# Autodesk Inventor assembly: Gripper_Design_Non_Compliant_v1
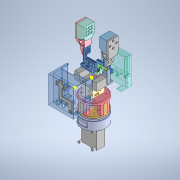
[picture p0: Inventor's stored thumbnail of the model, 180x180]
Saved by Autodesk Inventor 2022 (Build 260153000, 153)
## iProperties
Created: 2021-07-25
Part Number: Gripper_Design_Non_Compliant_v1
Document SubType Name: Assembly
Designer: exllu
Author: exllu
## Documents named in this file (36)
- C:\Users\kylem\OneDrive\Documents\1 - Documents\Gripper Design\Gripper_Design_Non_Compliant_v1.iam
- C:\Users\kylem\OneDrive\Documents\1 - Documents\Gripper Design\Motor_XM,H-430_idler.ipt
- C:\Users\kylem\OneDrive\Documents\1 - Documents\Gripper Design\Carriage_8381K550.iam
- C:\Users\kylem\OneDrive\Documents\1 - Documents\Gripper Design\Rail_8381K550.iam
- C:\Users\kylem\OneDrive\Documents\1 - Documents\Gripper Design\Pinion_2664N316.ipt
- C:\Users\kylem\OneDrive\Documents\1 - Documents\Gripper Design\Drive_shaft.ipt
- C:\Users\kylem\OneDrive\Documents\1 - Documents\Gripper Design\Motor_horn_mount.ipt
- C:\Users\kylem\OneDrive\Documents\1 - Documents\Gripper Design\Rack.iam
- C:\Users\kylem\OneDrive\Documents\1 - Documents\Gripper Design\UR5 Robot\End-effector-plate.ipt
- C:\Users\kylem\OneDrive\Documents\1 - Documents\Gripper Design\Rail_lock_washer.ipt
- C:\Users\exllu\Downloads\Rail_nut.ipt
- C:\Users\exllu\Downloads\90910A901_Button Head Torx Screws.ipt
- C:\Users\kylem\OneDrive\Documents\1 - Documents\Gripper Design\Rail_screws.ipt
- C:\Users\kylem\OneDrive\Documents\1 - Documents\Gripper Design\Rail_mount.ipt
- C:\Users\kylem\OneDrive\Documents\1 - Documents\Gripper Design\Front_plate.ipt
- C:\Users\exllu\Downloads\UR5_Screws.ipt
- C:\Users\kylem\OneDrive\Documents\1 - Documents\Gripper Design\UR5_Mounting_Plate.ipt
- C:\Users\kylem\OneDrive\Documents\1 - Documents\Gripper Design\Motor_UR5_mount.ipt
- C:\Users\kylem\OneDrive\Documents\1 - Documents\Gripper Design\Cover_bottom.ipt
- C:\Users\kylem\OneDrive\Documents\1 - Documents\Gripper Design\Cover_top.ipt
- C:\Users\kylem\OneDrive\Documents\1 - Documents\Gripper Design\Non_compliant_plate.ipt
- C:\Users\kylem\OneDrive\Documents\1 - Documents\Gripper Design\Cover_bottom_raceway_cover.ipt
- C:\Users\exllu\Downloads\98689A110_ METRIC GENERAL PURPOSE WASHERS.ipt
- C:\Users\exllu\Downloads\91292A004_TYPE 18-8 SS SOCKET HEAD CAP SCREW.ipt
- C:\Users\exllu\Downloads\98689A112_ METRIC GENERAL PURPOSE WASHERS.ipt
- C:\Users\exllu\Downloads\92855A309_18-8 Stainless Steel Low-Profile Socket Head Screws.ipt
- C:\Users\exllu\Downloads\97163A149_TAPERED HEAT-SET INSERTS FOR PLASTIC .ipt
- C:\Users\exllu\Downloads\91223A411_316 SS ULTRA-LOW-PROFILE SOCKET HEAD SCREW.ipt
- C:\Users\exllu\Downloads\91290A099_Black-Oxide Alloy Steel Socket Head Screw.ipt
- C:\Users\exllu\Downloads\91292A834_TYPE 18-8 SS SOCKET HEAD CAP SCREW.ipt
- C:\Users\exllu\Downloads\91292A016_TYPE 18-8 SS SOCKET HEAD CAP SCREW.ipt
- C:\Users\exllu\Downloads\91292A022_18-8 Stainless Steel Socket Head Screw.ipt
- C:\Users\exllu\Downloads\97400A135_18-8 STAINLESS STEEL SERRATED FLANGE LOCKNUT.ipt
- C:\Users\kylem\OneDrive\Documents\1 - Documents\Gripper Design\U2D2PHB_Board.ipt
- C:\Users\kylem\OneDrive\Documents\1 - Documents\Gripper Design\Finger Assembly Left.iam
- C:\Users\kylem\OneDrive\Documents\1 - Documents\Gripper Design\Finger Assembly Right.iam
## Components (86 placed, 35 different names)
1. Motor_XM,H-430_idler:1 — Flush:1, Flush:2, Flush:3, Flush:7, Mate:15, Mate:16, Mate:29, Flush:22, Mate:65, Flush:33, Flush:34, Mate:132, Mate:218, Mate:238
2. Rail_8381K550:3 [sub-assembly] — Mate:3, Mate:4, Mate:5, Mate:6, Flush:7, Mate:29, Mate:30, Flush:18, Flush:19, Mate:36, Mate:40, Mate:41, Mate:44, Mate:45, Mate:47, Mate:53, Mate:55, Mate:56, Mate:57, Mate:59, Mate:61, Mate:62, Flush:25
3. Rail_8381K550:4 [sub-assembly] — Mate:1, Mate:2, Mate:7, Mate:8, Mate:30, Flush:18, Flush:19, Mate:32, Mate:33, Mate:34, Mate:35, Mate:37, Mate:38, Mate:39, Mate:46, Mate:63
4. Carriage_8381K550:5 [sub-assembly] — Mate:4, Mate:5, Flush:12, Mate:137, Mate:138, Mate:139, Mate:142
5. Carriage_8381K550:6 [sub-assembly] — Mate:1, Mate:7, Mate:13, Mate:140, Mate:143
6. Carriage_8381K550:7 [sub-assembly] — Mate:3, Mate:6, Mate:142
7. Carriage_8381K550:8 [sub-assembly] — Mate:2, Mate:8, Mate:13, Flush:23, Mate:141
8. Pinion_2664N316:1 — Mate:20, Mate:21, Flush:20, Tangent:1, Tangent:2, Rotation/Translation:1, Rotation/Translation:2, Mate:240
9. Drive_shaft:1 — Mate:17, Mate:20, Mate:21, Mate:66, Mate:220, Mate:221
10. Motor_horn_mount:1 — Mate:15, Mate:16, Mate:17, Mate:64, Mate:66
11. Rack:1 [sub-assembly] — Flush:20, Tangent:1, Flush:23, Rotation/Translation:2, Mate:190, Mate:191, Mate:192
12. Rack:2 [sub-assembly] — Flush:12, Tangent:2, Rotation/Translation:1, Mate:182, Mate:185, Mate:186
13. End-effector-plate:1 — Flush:33, Flush:34, Mate:111, Mate:126, Mate:133
14. Rail_lock_washer:1 — Mate:40, Mate:41, Mate:52
15. Rail_nut:1 — Mate:32, Mate:39
16. Rail_nut:2 — Mate:33, Mate:38
17. Rail_lock_washer:3 — Mate:44, Mate:47, Mate:54
18. Rail_nut:3 — Mate:34, Mate:37
19. Rail_lock_washer:4 — Mate:45, Mate:46, Mate:60
20. Rail_nut:4 — Mate:35, Mate:36
21. 90910A901_Button Head Torx Screws:1 — Mate:52, Mate:53
22. Rail_screws:1 — Mate:60, Mate:61
23. Rail_screws:2 — Mate:54, Mate:55
24. Rail_screws:3 — Mate:58, Mate:59
25. Rail_lock_washer:5 — Mate:56, Mate:57, Mate:58
26. Rail_mount:1 — Mate:62, Mate:63, Flush:25, Mate:68, Mate:135, Mate:209
27. Front_plate:1 — Flush:22, Mate:64, Mate:65, Mate:68, Mate:210, Mate:222, Mate:223, Mate:240
28. UR5_Screws:1 — Mate:114, Mate:115
29. UR5_Screws:3 — Mate:118, Mate:122
30. UR5_Screws:4 — Mate:112, Mate:124
31. UR5_Mounting_Plate:1 — Mate:111, Mate:112, Mate:114, Mate:115, Mate:118, Mate:122, Mate:124, Mate:126, Mate:127, Mate:128, Mate:129, Mate:131, Mate:133
32. Motor_UR5_mount:1 — Mate:129, Mate:131, Mate:132, Mate:134, Mate:136, Mate:224, Mate:225, Mate:228, Mate:229, Mate:232, Mate:234, Mate:236, Mate:237
33. UR5_Screws:5 — Mate:127, Mate:128
34. Cover_bottom:1 — Mate:134, Mate:135, Flush:35, Mate:145, Flush:36, Mate:146, Flush:41, Mate:214, Mate:239
35. Cover_top:1 — Mate:136, Flush:35, Mate:216, Mate:217, Mate:219
36. Non_compliant_plate:1 — Mate:140, Mate:141, Mate:143, Mate:155, Mate:156, Mate:157, Mate:158, Mate:159, Mate:160, Mate:161, Mate:162, Mate:173, Mate:174, Mate:175, Mate:176, Mate:187, Mate:188, Mate:189, Mate:207, Mate:208, Flush:39, Flush:40, Mate:242, Flush:42, Mate:244
37. Non_compliant_plate:2 — Mate:137, Mate:138, Mate:139, Mate:147, Mate:148, Mate:149, Mate:150, Mate:151, Mate:152, Mate:153, Mate:154, Mate:177, Mate:178, Mate:179, Mate:180, Mate:181, Mate:183, Mate:184, Mate:205, Mate:206, Flush:37, Flush:38, Mate:241, Flush:43, Mate:243
38. Cover_bottom_raceway_cover:1 — Mate:145, Flush:36, Mate:146, Mate:211, Mate:212
39. 98689A110_ METRIC GENERAL PURPOSE WASHERS:1 — Mate:149, Mate:152, Mate:166
40. 98689A110_ METRIC GENERAL PURPOSE WASHERS:2 — Mate:158, Mate:159, Mate:172
41. 98689A110_ METRIC GENERAL PURPOSE WASHERS:3 — Mate:156, Mate:161, Mate:170
42. 98689A110_ METRIC GENERAL PURPOSE WASHERS:4 — Mate:157, Mate:160, Mate:171
43. 98689A110_ METRIC GENERAL PURPOSE WASHERS:5 — Mate:155, Mate:162, Mate:169
44. 98689A110_ METRIC GENERAL PURPOSE WASHERS:6 — Mate:150, Mate:151, Mate:165
45. 98689A110_ METRIC GENERAL PURPOSE WASHERS:7 — Mate:147, Mate:154, Mate:168
46. 98689A110_ METRIC GENERAL PURPOSE WASHERS:8 — Mate:148, Mate:153, Mate:167
47. 91292A004_TYPE 18-8 SS SOCKET HEAD CAP SCREW:1 — Mate:168, Mate:180
48. 91292A004_TYPE 18-8 SS SOCKET HEAD CAP SCREW:2 — Mate:166, Mate:178
49. 91292A004_TYPE 18-8 SS SOCKET HEAD CAP SCREW:3 — Mate:165, Mate:177
50. 91292A004_TYPE 18-8 SS SOCKET HEAD CAP SCREW:4 — Mate:167, Mate:179
51. 91292A004_TYPE 18-8 SS SOCKET HEAD CAP SCREW:5 — Mate:171, Mate:174
52. 91292A004_TYPE 18-8 SS SOCKET HEAD CAP SCREW:6 — Mate:169, Mate:176
53. 91292A004_TYPE 18-8 SS SOCKET HEAD CAP SCREW:7 — Mate:172, Mate:173
54. 91292A004_TYPE 18-8 SS SOCKET HEAD CAP SCREW:8 — Mate:170, Mate:175
55. 98689A112_ METRIC GENERAL PURPOSE WASHERS:1 — Mate:181, Mate:182, Mate:193, Mate:204
56. 98689A112_ METRIC GENERAL PURPOSE WASHERS:2 — Mate:189, Mate:191, Mate:197, Mate:200
57. 98689A112_ METRIC GENERAL PURPOSE WASHERS:3 — Mate:188, Mate:190, Mate:196, Mate:201
58. 98689A112_ METRIC GENERAL PURPOSE WASHERS:4 — Mate:187, Mate:192, Mate:198, Mate:199
59. 98689A112_ METRIC GENERAL PURPOSE WASHERS:6 — Mate:184, Mate:186, Mate:195, Mate:202
60. 98689A112_ METRIC GENERAL PURPOSE WASHERS:7 — Mate:183, Mate:185, Mate:194, Mate:203
61. 92855A309_18-8 Stainless Steel Low-Profile Socket Head Screws:1 — Mate:195, Mate:202
62. 92855A309_18-8 Stainless Steel Low-Profile Socket Head Screws:2 — Mate:198, Mate:199
63. 92855A309_18-8 Stainless Steel Low-Profile Socket Head Screws:3 — Mate:194, Mate:203
64. 92855A309_18-8 Stainless Steel Low-Profile Socket Head Screws:4 — Mate:197, Mate:200
65. 92855A309_18-8 Stainless Steel Low-Profile Socket Head Screws:5 — Mate:193, Mate:204
66. 92855A309_18-8 Stainless Steel Low-Profile Socket Head Screws:6 — Mate:196, Mate:201
67. 97163A149_TAPERED HEAT-SET INSERTS FOR PLASTIC :1 — Mate:205, Flush:38
68. 97163A149_TAPERED HEAT-SET INSERTS FOR PLASTIC :2 — Mate:206, Flush:37
69. 97163A149_TAPERED HEAT-SET INSERTS FOR PLASTIC :3 — Mate:207, Flush:40
70. 97163A149_TAPERED HEAT-SET INSERTS FOR PLASTIC :4 — Mate:208, Flush:39
71. 92855A309_18-8 Stainless Steel Low-Profile Socket Head Screws:7 — Mate:209, Mate:210
72. 91223A411_316 SS ULTRA-LOW-PROFILE SOCKET HEAD SCREW:1 — Mate:211, Mate:212
73. 97163A149_TAPERED HEAT-SET INSERTS FOR PLASTIC :5 — Flush:41, Mate:214
74. 92855A309_18-8 Stainless Steel Low-Profile Socket Head Screws:8 — Mate:216, Mate:217
75. 91290A099_Black-Oxide Alloy Steel Socket Head Screw:1 — Mate:218, Mate:219
76. 91292A834_TYPE 18-8 SS SOCKET HEAD CAP SCREW:1 — Mate:220, Mate:221
77. 91292A016_TYPE 18-8 SS SOCKET HEAD CAP SCREW:1 — Mate:222, Mate:223
78. 91292A022_18-8 Stainless Steel Socket Head Screw:1 — Mate:224, Mate:225, Mate:233
79. 91292A022_18-8 Stainless Steel Socket Head Screw:2 — Mate:228, Mate:229, Mate:235
80. 97400A135_18-8 STAINLESS STEEL SERRATED FLANGE LOCKNUT:1 — Mate:232, Mate:233
81. 97400A135_18-8 STAINLESS STEEL SERRATED FLANGE LOCKNUT:2 — Mate:234, Mate:235
82. 91292A016_TYPE 18-8 SS SOCKET HEAD CAP SCREW:2 — Mate:236, Mate:237
83. 91290A099_Black-Oxide Alloy Steel Socket Head Screw:2 — Mate:238, Mate:239
84. U2D2PHB_Board:1
85. Finger Assembly Left:1 [sub-assembly] — Mate:241, Flush:43, Mate:243
86. Finger Assembly Right:1 [sub-assembly] — Mate:242, Flush:42, Mate:244
## Relationships (188: Mate 162, Flush 22, Tangent 2, RelateRotateTranslate 2)
- Mate:1 (0.1 mm): Rail_8381K550:4 ↔ Carriage_8381K550:6
- Mate:2 (0.1 mm): Rail_8381K550:4 ↔ Carriage_8381K550:8
- Mate:3 (0.1 mm): Rail_8381K550:3 ↔ Carriage_8381K550:7
- Mate:4 (0.1 mm): Rail_8381K550:3 ↔ Carriage_8381K550:5
- Mate:5 (0.2 mm): Rail_8381K550:3 ↔ Carriage_8381K550:5
- Mate:6 (0.2 mm): Rail_8381K550:3 ↔ Carriage_8381K550:7
- Mate:7 (0.2 mm): Rail_8381K550:4 ↔ Carriage_8381K550:6
- Mate:8 (0.2 mm): Rail_8381K550:4 ↔ Carriage_8381K550:8
- Flush:1: Motor_XM,H-430_idler:1
- Flush:2: Motor_XM,H-430_idler:1
- Flush:3: Motor_XM,H-430_idler:1
- Mate:13: Carriage_8381K550:6 ↔ Carriage_8381K550:8
- Flush:7 (-20.75 mm): Motor_XM,H-430_idler:1 ↔ Rail_8381K550:3
- Mate:15: Motor_XM,H-430_idler:1 ↔ Motor_horn_mount:1
- Mate:16: Motor_XM,H-430_idler:1 ↔ Motor_horn_mount:1
- Mate:17: Drive_shaft:1 ↔ Motor_horn_mount:1
- Mate:20: Pinion_2664N316:1 ↔ Drive_shaft:1
- Mate:21: Pinion_2664N316:1 ↔ Drive_shaft:1
- Flush:12: Carriage_8381K550:5 ↔ Rack:2
- Mate:29 (-10.75 mm): Motor_XM,H-430_idler:1 ↔ Rail_8381K550:3
- Mate:30 (1 mm): Rail_8381K550:3 ↔ Rail_8381K550:4
- Flush:18: Rail_8381K550:3 ↔ Rail_8381K550:4
- Flush:19: Rail_8381K550:3 ↔ Rail_8381K550:4
- Flush:20: Pinion_2664N316:1 ↔ Rack:1
- Mate:32: Rail_8381K550:4 ↔ Rail_nut:1
- Mate:33: Rail_8381K550:4 ↔ Rail_nut:2
- Mate:34: Rail_8381K550:4 ↔ Rail_nut:3
- Mate:35: Rail_8381K550:4 ↔ Rail_nut:4
- Mate:36: Rail_8381K550:3 ↔ Rail_nut:4
- Mate:37: Rail_8381K550:4 ↔ Rail_nut:3
- Mate:38: Rail_8381K550:4 ↔ Rail_nut:2
- Mate:39: Rail_8381K550:4 ↔ Rail_nut:1
- Mate:40: Rail_8381K550:3 ↔ Rail_lock_washer:1
- Mate:41: Rail_8381K550:3 ↔ Rail_lock_washer:1
- Mate:44: Rail_8381K550:3 ↔ Rail_lock_washer:3
- Mate:45: Rail_8381K550:3 ↔ Rail_lock_washer:4
- Mate:46: Rail_8381K550:4 ↔ Rail_lock_washer:4
- Mate:47: Rail_8381K550:3 ↔ Rail_lock_washer:3
- Mate:52: Rail_lock_washer:1 ↔ 90910A901_Button Head Torx Screws:1
- Mate:53: Rail_8381K550:3 ↔ 90910A901_Button Head Torx Screws:1
- Mate:54: Rail_lock_washer:3 ↔ Rail_screws:2
- Mate:55: Rail_8381K550:3 ↔ Rail_screws:2
- Mate:56: Rail_8381K550:3 ↔ Rail_lock_washer:5
- Mate:57: Rail_8381K550:3 ↔ Rail_lock_washer:5
- Mate:58: Rail_screws:3 ↔ Rail_lock_washer:5
- Mate:59: Rail_8381K550:3 ↔ Rail_screws:3
- Mate:60: Rail_lock_washer:4 ↔ Rail_screws:1
- Mate:61: Rail_8381K550:3 ↔ Rail_screws:1
- Mate:62: Rail_8381K550:3 ↔ Rail_mount:1
- Mate:63: Rail_8381K550:4 ↔ Rail_mount:1
- Flush:22: Motor_XM,H-430_idler:1 ↔ Front_plate:1
- Mate:64: Motor_horn_mount:1 ↔ Front_plate:1
- Mate:65: Motor_XM,H-430_idler:1 ↔ Front_plate:1
- Tangent:1 (-1 mm): Pinion_2664N316:1 ↔ Rack:1
- Tangent:2 (-1 mm): Pinion_2664N316:1 ↔ Rack:2
- Rotation/Translation:1 [RelateRotateTranslate] (39.841 mm): Pinion_2664N316:1 ↔ Rack:2
- Mate:66: Drive_shaft:1 ↔ Motor_horn_mount:1
- Flush:23: Carriage_8381K550:8 ↔ Rack:1
- Flush:25: Rail_8381K550:3 ↔ Rail_mount:1
- Mate:68: Rail_mount:1 ↔ Front_plate:1
- Rotation/Translation:2 [RelateRotateTranslate] (40.841 mm): Pinion_2664N316:1 ↔ Rack:1
- Flush:33 (4.572 mm): Motor_XM,H-430_idler:1 ↔ End-effector-plate:1
- Flush:34 (15.25 mm): Motor_XM,H-430_idler:1 ↔ End-effector-plate:1
- Mate:111: End-effector-plate:1 ↔ UR5_Mounting_Plate:1
- Mate:112: UR5_Screws:4 ↔ UR5_Mounting_Plate:1
- Mate:114: UR5_Screws:1 ↔ UR5_Mounting_Plate:1
- Mate:115: UR5_Screws:1 ↔ UR5_Mounting_Plate:1
- Mate:118: UR5_Screws:3 ↔ UR5_Mounting_Plate:1
- Mate:122: UR5_Screws:3 ↔ UR5_Mounting_Plate:1
- Mate:124: UR5_Screws:4 ↔ UR5_Mounting_Plate:1
- Mate:126: End-effector-plate:1 ↔ UR5_Mounting_Plate:1
- Mate:127: UR5_Mounting_Plate:1 ↔ UR5_Screws:5
- Mate:128: UR5_Mounting_Plate:1 ↔ UR5_Screws:5
- Mate:129: UR5_Mounting_Plate:1 ↔ Motor_UR5_mount:1
- Mate:131: UR5_Mounting_Plate:1 ↔ Motor_UR5_mount:1
- Mate:132: Motor_XM,H-430_idler:1 ↔ Motor_UR5_mount:1
- Mate:133: End-effector-plate:1 ↔ UR5_Mounting_Plate:1
- Mate:134: Motor_UR5_mount:1 ↔ Cover_bottom:1
- Mate:135 (0.5 mm): Rail_mount:1 ↔ Cover_bottom:1
- Mate:136: Motor_UR5_mount:1 ↔ Cover_top:1
- Flush:35: Cover_bottom:1 ↔ Cover_top:1
- Mate:137: Carriage_8381K550:5 ↔ Non_compliant_plate:2
- Mate:138: Carriage_8381K550:5 ↔ Non_compliant_plate:2
- Mate:139: Carriage_8381K550:5 ↔ Non_compliant_plate:2
- Mate:140: Carriage_8381K550:6 ↔ Non_compliant_plate:1
- Mate:141: Carriage_8381K550:8 ↔ Non_compliant_plate:1
- Mate:142: Carriage_8381K550:5 ↔ Carriage_8381K550:7
- Mate:143: Carriage_8381K550:6 ↔ Non_compliant_plate:1
- Mate:145: Cover_bottom:1 ↔ Cover_bottom_raceway_cover:1
- Flush:36: Cover_bottom:1 ↔ Cover_bottom_raceway_cover:1
- Mate:146: Cover_bottom:1 ↔ Cover_bottom_raceway_cover:1
- Mate:147: Non_compliant_plate:2 ↔ 98689A110_ METRIC GENERAL PURPOSE WASHERS:7
- Mate:148: Non_compliant_plate:2 ↔ 98689A110_ METRIC GENERAL PURPOSE WASHERS:8
- Mate:149: Non_compliant_plate:2 ↔ 98689A110_ METRIC GENERAL PURPOSE WASHERS:1
- Mate:150: Non_compliant_plate:2 ↔ 98689A110_ METRIC GENERAL PURPOSE WASHERS:6
- Mate:151: Non_compliant_plate:2 ↔ 98689A110_ METRIC GENERAL PURPOSE WASHERS:6
- Mate:152: Non_compliant_plate:2 ↔ 98689A110_ METRIC GENERAL PURPOSE WASHERS:1
- Mate:153: Non_compliant_plate:2 ↔ 98689A110_ METRIC GENERAL PURPOSE WASHERS:8
- Mate:154: Non_compliant_plate:2 ↔ 98689A110_ METRIC GENERAL PURPOSE WASHERS:7
- Mate:155: Non_compliant_plate:1 ↔ 98689A110_ METRIC GENERAL PURPOSE WASHERS:5
- Mate:156: Non_compliant_plate:1 ↔ 98689A110_ METRIC GENERAL PURPOSE WASHERS:3
- Mate:157: Non_compliant_plate:1 ↔ 98689A110_ METRIC GENERAL PURPOSE WASHERS:4
- Mate:158: Non_compliant_plate:1 ↔ 98689A110_ METRIC GENERAL PURPOSE WASHERS:2
- Mate:159: Non_compliant_plate:1 ↔ 98689A110_ METRIC GENERAL PURPOSE WASHERS:2
- Mate:160: Non_compliant_plate:1 ↔ 98689A110_ METRIC GENERAL PURPOSE WASHERS:4
- Mate:161: Non_compliant_plate:1 ↔ 98689A110_ METRIC GENERAL PURPOSE WASHERS:3
- Mate:162: Non_compliant_plate:1 ↔ 98689A110_ METRIC GENERAL PURPOSE WASHERS:5
- Mate:165: 98689A110_ METRIC GENERAL PURPOSE WASHERS:6 ↔ 91292A004_TYPE 18-8 SS SOCKET HEAD CAP SCREW:3
- Mate:166: 98689A110_ METRIC GENERAL PURPOSE WASHERS:1 ↔ 91292A004_TYPE 18-8 SS SOCKET HEAD CAP SCREW:2
- Mate:167: 98689A110_ METRIC GENERAL PURPOSE WASHERS:8 ↔ 91292A004_TYPE 18-8 SS SOCKET HEAD CAP SCREW:4
- Mate:168: 98689A110_ METRIC GENERAL PURPOSE WASHERS:7 ↔ 91292A004_TYPE 18-8 SS SOCKET HEAD CAP SCREW:1
- Mate:169: 98689A110_ METRIC GENERAL PURPOSE WASHERS:5 ↔ 91292A004_TYPE 18-8 SS SOCKET HEAD CAP SCREW:6
- Mate:170: 98689A110_ METRIC GENERAL PURPOSE WASHERS:3 ↔ 91292A004_TYPE 18-8 SS SOCKET HEAD CAP SCREW:8
- Mate:171: 98689A110_ METRIC GENERAL PURPOSE WASHERS:4 ↔ 91292A004_TYPE 18-8 SS SOCKET HEAD CAP SCREW:5
- Mate:172: 98689A110_ METRIC GENERAL PURPOSE WASHERS:2 ↔ 91292A004_TYPE 18-8 SS SOCKET HEAD CAP SCREW:7
- Mate:173: Non_compliant_plate:1 ↔ 91292A004_TYPE 18-8 SS SOCKET HEAD CAP SCREW:7
- Mate:174: Non_compliant_plate:1 ↔ 91292A004_TYPE 18-8 SS SOCKET HEAD CAP SCREW:5
- Mate:175: Non_compliant_plate:1 ↔ 91292A004_TYPE 18-8 SS SOCKET HEAD CAP SCREW:8
- Mate:176: Non_compliant_plate:1 ↔ 91292A004_TYPE 18-8 SS SOCKET HEAD CAP SCREW:6
- Mate:177: Non_compliant_plate:2 ↔ 91292A004_TYPE 18-8 SS SOCKET HEAD CAP SCREW:3
- Mate:178: Non_compliant_plate:2 ↔ 91292A004_TYPE 18-8 SS SOCKET HEAD CAP SCREW:2
- Mate:179: Non_compliant_plate:2 ↔ 91292A004_TYPE 18-8 SS SOCKET HEAD CAP SCREW:4
- Mate:180: Non_compliant_plate:2 ↔ 91292A004_TYPE 18-8 SS SOCKET HEAD CAP SCREW:1
- Mate:181: Non_compliant_plate:2 ↔ 98689A112_ METRIC GENERAL PURPOSE WASHERS:1
- Mate:182: Rack:2 ↔ 98689A112_ METRIC GENERAL PURPOSE WASHERS:1
- Mate:183: Non_compliant_plate:2 ↔ 98689A112_ METRIC GENERAL PURPOSE WASHERS:7
- Mate:184: Non_compliant_plate:2 ↔ 98689A112_ METRIC GENERAL PURPOSE WASHERS:6
- Mate:185: Rack:2 ↔ 98689A112_ METRIC GENERAL PURPOSE WASHERS:7
- Mate:186: Rack:2 ↔ 98689A112_ METRIC GENERAL PURPOSE WASHERS:6
- Mate:187: Non_compliant_plate:1 ↔ 98689A112_ METRIC GENERAL PURPOSE WASHERS:4
- Mate:188: Non_compliant_plate:1 ↔ 98689A112_ METRIC GENERAL PURPOSE WASHERS:3
- Mate:189: Non_compliant_plate:1 ↔ 98689A112_ METRIC GENERAL PURPOSE WASHERS:2
- Mate:190: Rack:1 ↔ 98689A112_ METRIC GENERAL PURPOSE WASHERS:3
- Mate:191: Rack:1 ↔ 98689A112_ METRIC GENERAL PURPOSE WASHERS:2
- Mate:192: Rack:1 ↔ 98689A112_ METRIC GENERAL PURPOSE WASHERS:4
- Mate:193: 98689A112_ METRIC GENERAL PURPOSE WASHERS:1 ↔ 92855A309_18-8 Stainless Steel Low-Profile Socket Head Screws:5
- Mate:194: 98689A112_ METRIC GENERAL PURPOSE WASHERS:7 ↔ 92855A309_18-8 Stainless Steel Low-Profile Socket Head Screws:3
- Mate:195: 98689A112_ METRIC GENERAL PURPOSE WASHERS:6 ↔ 92855A309_18-8 Stainless Steel Low-Profile Socket Head Screws:1
- Mate:196: 98689A112_ METRIC GENERAL PURPOSE WASHERS:3 ↔ 92855A309_18-8 Stainless Steel Low-Profile Socket Head Screws:6
- Mate:197: 98689A112_ METRIC GENERAL PURPOSE WASHERS:2 ↔ 92855A309_18-8 Stainless Steel Low-Profile Socket Head Screws:4
- Mate:198: 98689A112_ METRIC GENERAL PURPOSE WASHERS:4 ↔ 92855A309_18-8 Stainless Steel Low-Profile Socket Head Screws:2
- Mate:199: 98689A112_ METRIC GENERAL PURPOSE WASHERS:4 ↔ 92855A309_18-8 Stainless Steel Low-Profile Socket Head Screws:2
- Mate:200: 98689A112_ METRIC GENERAL PURPOSE WASHERS:2 ↔ 92855A309_18-8 Stainless Steel Low-Profile Socket Head Screws:4
- Mate:201: 98689A112_ METRIC GENERAL PURPOSE WASHERS:3 ↔ 92855A309_18-8 Stainless Steel Low-Profile Socket Head Screws:6
- Mate:202: 98689A112_ METRIC GENERAL PURPOSE WASHERS:6 ↔ 92855A309_18-8 Stainless Steel Low-Profile Socket Head Screws:1
- Mate:203: 98689A112_ METRIC GENERAL PURPOSE WASHERS:7 ↔ 92855A309_18-8 Stainless Steel Low-Profile Socket Head Screws:3
- Mate:204: 98689A112_ METRIC GENERAL PURPOSE WASHERS:1 ↔ 92855A309_18-8 Stainless Steel Low-Profile Socket Head Screws:5
- Mate:205: Non_compliant_plate:2 ↔ 97163A149_TAPERED HEAT-SET INSERTS FOR PLASTIC :1
- Mate:206: Non_compliant_plate:2 ↔ 97163A149_TAPERED HEAT-SET INSERTS FOR PLASTIC :2
- Flush:37: Non_compliant_plate:2 ↔ 97163A149_TAPERED HEAT-SET INSERTS FOR PLASTIC :2
- Flush:38: Non_compliant_plate:2 ↔ 97163A149_TAPERED HEAT-SET INSERTS FOR PLASTIC :1
- Mate:207: Non_compliant_plate:1 ↔ 97163A149_TAPERED HEAT-SET INSERTS FOR PLASTIC :3
- Mate:208: Non_compliant_plate:1 ↔ 97163A149_TAPERED HEAT-SET INSERTS FOR PLASTIC :4
- Flush:39: Non_compliant_plate:1 ↔ 97163A149_TAPERED HEAT-SET INSERTS FOR PLASTIC :4
- Flush:40: Non_compliant_plate:1 ↔ 97163A149_TAPERED HEAT-SET INSERTS FOR PLASTIC :3
- Mate:209: Rail_mount:1 ↔ 92855A309_18-8 Stainless Steel Low-Profile Socket Head Screws:7
- Mate:210: Front_plate:1 ↔ 92855A309_18-8 Stainless Steel Low-Profile Socket Head Screws:7
- Mate:211: Cover_bottom_raceway_cover:1 ↔ 91223A411_316 SS ULTRA-LOW-PROFILE SOCKET HEAD SCREW:1
- Mate:212: Cover_bottom_raceway_cover:1 ↔ 91223A411_316 SS ULTRA-LOW-PROFILE SOCKET HEAD SCREW:1
- Flush:41: Cover_bottom:1 ↔ 97163A149_TAPERED HEAT-SET INSERTS FOR PLASTIC :5
- Mate:214: Cover_bottom:1 ↔ 97163A149_TAPERED HEAT-SET INSERTS FOR PLASTIC :5
- Mate:216: Cover_top:1 ↔ 92855A309_18-8 Stainless Steel Low-Profile Socket Head Screws:8
- Mate:217: Cover_top:1 ↔ 92855A309_18-8 Stainless Steel Low-Profile Socket Head Screws:8
- Mate:218: Motor_XM,H-430_idler:1 ↔ 91290A099_Black-Oxide Alloy Steel Socket Head Screw:1
- Mate:219: Cover_top:1 ↔ 91290A099_Black-Oxide Alloy Steel Socket Head Screw:1
- Mate:220: Drive_shaft:1 ↔ 91292A834_TYPE 18-8 SS SOCKET HEAD CAP SCREW:1
- Mate:221: Drive_shaft:1 ↔ 91292A834_TYPE 18-8 SS SOCKET HEAD CAP SCREW:1
- Mate:222: Front_plate:1 ↔ 91292A016_TYPE 18-8 SS SOCKET HEAD CAP SCREW:1
- Mate:223: Front_plate:1 ↔ 91292A016_TYPE 18-8 SS SOCKET HEAD CAP SCREW:1
- Mate:224: Motor_UR5_mount:1 ↔ 91292A022_18-8 Stainless Steel Socket Head Screw:1
- Mate:225: Motor_UR5_mount:1 ↔ 91292A022_18-8 Stainless Steel Socket Head Screw:1
- Mate:228: Motor_UR5_mount:1 ↔ 91292A022_18-8 Stainless Steel Socket Head Screw:2
- Mate:229: Motor_UR5_mount:1 ↔ 91292A022_18-8 Stainless Steel Socket Head Screw:2
- Mate:232: Motor_UR5_mount:1 ↔ 97400A135_18-8 STAINLESS STEEL SERRATED FLANGE LOCKNUT:1
- Mate:233: 91292A022_18-8 Stainless Steel Socket Head Screw:1 ↔ 97400A135_18-8 STAINLESS STEEL SERRATED FLANGE LOCKNUT:1
- Mate:234: Motor_UR5_mount:1 ↔ 97400A135_18-8 STAINLESS STEEL SERRATED FLANGE LOCKNUT:2
- Mate:235: 91292A022_18-8 Stainless Steel Socket Head Screw:2 ↔ 97400A135_18-8 STAINLESS STEEL SERRATED FLANGE LOCKNUT:2
- Mate:236: Motor_UR5_mount:1 ↔ 91292A016_TYPE 18-8 SS SOCKET HEAD CAP SCREW:2
- Mate:237: Motor_UR5_mount:1 ↔ 91292A016_TYPE 18-8 SS SOCKET HEAD CAP SCREW:2
- Mate:238: Motor_XM,H-430_idler:1 ↔ 91290A099_Black-Oxide Alloy Steel Socket Head Screw:2
- Mate:239: Cover_bottom:1 ↔ 91290A099_Black-Oxide Alloy Steel Socket Head Screw:2
- Mate:240: Pinion_2664N316:1 ↔ Front_plate:1
- Mate:241: Non_compliant_plate:2 ↔ Finger Assembly Left:1
- Mate:242: Non_compliant_plate:1 ↔ Finger Assembly Right:1
- Flush:42: Non_compliant_plate:1 ↔ Finger Assembly Right:1
- Flush:43: Non_compliant_plate:2 ↔ Finger Assembly Left:1
- Mate:243: Non_compliant_plate:2 ↔ Finger Assembly Left:1
- Mate:244: Non_compliant_plate:1 ↔ Finger Assembly Right:1
